# Autodesk Inventor assembly: canaletaMedia
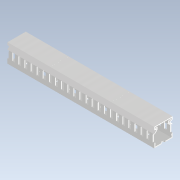
[picture p0: Inventor's stored thumbnail of the model, 180x180]
Saved by Autodesk Inventor 2021 (Build 250183000, 183)
## iProperties
Created: 2021-08-23
Part Number: canaletaMedia
Document SubType Name: Assembly
Designer: Andrés Holguín
Author: Andrés Holguín
## Documents named in this file (2)
- C:\Users\andre\Documents\GitHub\Dis.-Mecatronico-E6\inventor proyecto\Tablero\Canaletas\canaletaMedia.iam
- C:\Users\andre\Documents\GitHub\Dis.-Mecatronico-E6\inventor proyecto\Tablero\Canaletas\7308-1.iam
## Components (3 placed, 1 different names)
1. 7308-1:3 [sub-assembly] — Rigid:2, Mate:2, Angle:2, Mate:3, Angle:3
2. 7308-1:4 [sub-assembly] — Rigid:2, Rigid:3
3. 7308-1:5 [sub-assembly] — Rigid:3, Mate:1, Angle:1, Mate:4, Angle:4
## Relationships (10: Mate 4, Angle 4, WeldJoint 2)
- Rigid:2 [WeldJoint]: 7308-1:3 ↔ 7308-1:4
- Rigid:3 [WeldJoint]: 7308-1:4 ↔ 7308-1:5
- Mate:1: 7308-1:5
- Angle:1 (-45 deg): 7308-1:5
- Mate:2: 7308-1:3
- Angle:2 (-45 deg): 7308-1:3
- Mate:3: 7308-1:3
- Angle:3 (90 deg): 7308-1:3
- Mate:4: 7308-1:5
- Angle:4 (90 deg): 7308-1:5
